# Autodesk Inventor assembly: Shield
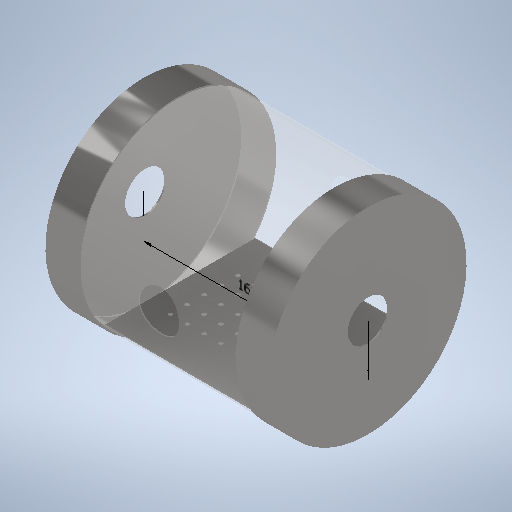
[picture p0: Inventor's stored thumbnail of the model, 512x512]
Saved by Autodesk Inventor 2025.3 (Build 293356000, 356)
## iProperties
Created: 2025-05-16
Part Number: Shield
Document SubType Name: Assembly
Designer: Verðandi
Author: Verðandi
## Documents named in this file (5)
- E:\Users\USER\Documents\GitHub\LAFriOC\Rb oven\MS-1L Shield\Shield.iam
- E:\Users\USER\Documents\GitHub\LAFriOC\Rb oven\MS-1L Shield\Shield Center.ipt
- E:\Users\USER\Documents\GitHub\LAFriOC\Rb oven\MS-1L Shield\Center Lid.ipt
- E:\Users\USER\Documents\GitHub\LAFriOC\Rb oven\MS-1L Shield\Center Lid_MIR.ipt
- E:\Users\USER\Documents\GitHub\LAFriOC\Rb oven\MS-1L Shield\Base.ipt
## Components (4 placed, 4 different names)
1. Shield Center:1 — Insert:1, Insert:3, Insert:4
2. Center Lid:1 — Insert:1
3. Center Lid_MIR:1 — Insert:4
4. Base:1 — Insert:3
## Relationships (3: Insert 3)
- Insert:1: Shield Center:1 ↔ Center Lid:1
- Insert:3 (-28 mm): Shield Center:1 ↔ Base:1
- Insert:4: Shield Center:1 ↔ Center Lid_MIR:1
